# Autodesk Inventor assembly: Ensamblaje_prueba
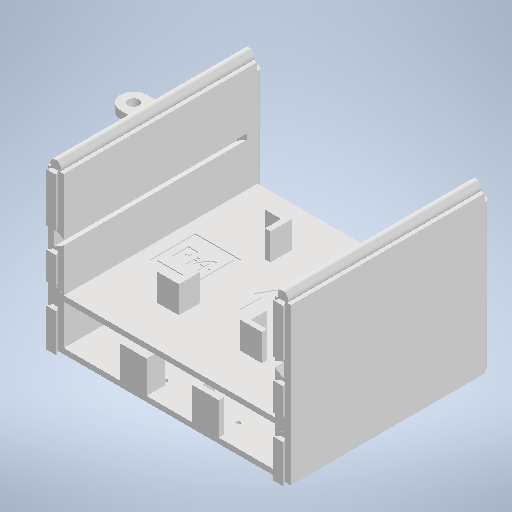
[picture p0: Inventor's stored thumbnail of the model, 512x512]
Saved by Autodesk Inventor 2025.1 (Build 291241000, 241)
## iProperties
Created: 2025-11-25
Part Number: Ensamblaje_prueba
Document SubType Name: Assembly
Designer: Diego
Author: Diego
## Documents named in this file (3)
- C:\Users\diego\OneDrive - Universidad de Oviedo\Uniovi\Master\2\CAVER\Inventor\Ensamblaje_prueba.iam
- C:\Users\diego\OneDrive - Universidad de Oviedo\Uniovi\Master\2\CAVER\Inventor\Piezas\Suelo.ipt
- C:\Users\diego\OneDrive - Universidad de Oviedo\Uniovi\Master\2\CAVER\Inventor\Piezas\Base_MIR.ipt
## Components (2 placed, 2 different names)
1. Base_MIR:1 — Corredera:1
2. Suelo:1 — Corredera:1
## Relationships (1: TranslationJoint 1)
- Corredera:1 [TranslationJoint]: Base_MIR:1 ↔ Suelo:1
